# Autodesk Inventor assembly: 2040-2040
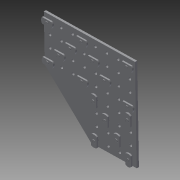
[picture p0: Inventor's stored thumbnail of the model, 180x180]
Saved by Autodesk Inventor 2014 (Build 180170000, 170)
## iProperties
Created: 2014-10-05
Part Number: 2040-2040
Document SubType Name: Assembly
Designer: Matthew
Author: Matthew
## Documents named in this file (3)
- C:\Users\Matthew\Documents\GitHub\CNC Mill\8020\2040-2040_right.iam
- C:\Users\Matthew\Documents\GitHub\CNC Mill\8020\2040-2040_mounting_plate.ipt
- C:\Users\Matthew\Documents\GitHub\CNC Mill\8020\0.5in_tnut.iam
## Components (17 placed, 2 different names)
1. 2040-2040_mounting_plate:1 — Insert:9, Insert:29, Insert:38, Insert:42, Insert:51, Insert:52, Insert:53, Insert:54, Insert:55, Insert:57, Insert:58, Insert:59, Insert:60, Insert:61, Insert:62, Insert:63
2. 0.5in_tnut:16 [sub-assembly] — Insert:9
3. 0.5in_tnut:28 [sub-assembly] — Insert:38
4. 0.5in_tnut:33 [sub-assembly] — Insert:42, Flush:1
5. 0.5in_tnut:44 [sub-assembly] — Insert:29, Flush:2
6. 0.5in_tnut:48 [sub-assembly] — Insert:51
7. 0.5in_tnut:52 [sub-assembly] — Insert:52, Flush:2
8. 0.5in_tnut:53 [sub-assembly] — Insert:53, Flush:1
9. 0.5in_tnut:54 [sub-assembly] — Insert:57
10. 0.5in_tnut:56 [sub-assembly] — Insert:55
11. 0.5in_tnut:57 [sub-assembly] — Insert:54
12. 0.5in_tnut:58 [sub-assembly] — Insert:59
13. 0.5in_tnut:59 [sub-assembly] — Insert:58
14. 0.5in_tnut:60 [sub-assembly] — Insert:60
15. 0.5in_tnut:61 [sub-assembly] — Insert:61
16. 0.5in_tnut:62 [sub-assembly] — Insert:62
17. 0.5in_tnut:63 [sub-assembly] — Insert:63
## Relationships (18: Insert 16, Flush 2)
- Insert:9: 2040-2040_mounting_plate:1 ↔ 0.5in_tnut:16
- Insert:29: 2040-2040_mounting_plate:1 ↔ 0.5in_tnut:44
- Insert:38: 2040-2040_mounting_plate:1 ↔ 0.5in_tnut:28
- Insert:42: 2040-2040_mounting_plate:1 ↔ 0.5in_tnut:33
- Insert:51: 2040-2040_mounting_plate:1 ↔ 0.5in_tnut:48
- Insert:52: 2040-2040_mounting_plate:1 ↔ 0.5in_tnut:52
- Insert:53: 2040-2040_mounting_plate:1 ↔ 0.5in_tnut:53
- Flush:1: 0.5in_tnut:33 ↔ 0.5in_tnut:53
- Flush:2: 0.5in_tnut:44 ↔ 0.5in_tnut:52
- Insert:54: 2040-2040_mounting_plate:1 ↔ 0.5in_tnut:57
- Insert:55: 2040-2040_mounting_plate:1 ↔ 0.5in_tnut:56
- Insert:57: 2040-2040_mounting_plate:1 ↔ 0.5in_tnut:54
- Insert:58: 2040-2040_mounting_plate:1 ↔ 0.5in_tnut:59
- Insert:59: 2040-2040_mounting_plate:1 ↔ 0.5in_tnut:58
- Insert:60: 2040-2040_mounting_plate:1 ↔ 0.5in_tnut:60
- Insert:61: 2040-2040_mounting_plate:1 ↔ 0.5in_tnut:61
- Insert:62: 2040-2040_mounting_plate:1 ↔ 0.5in_tnut:62
- Insert:63: 2040-2040_mounting_plate:1 ↔ 0.5in_tnut:63
